# Autodesk Inventor assembly: ModuloCocina
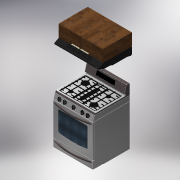
[picture p0: Inventor's stored thumbnail of the model, 180x180]
Saved by Autodesk Inventor 2016 (Build 200138000, 138)
## iProperties
Created: 2015-11-24
Part Number: ModuloCocina
Material: Genérico
Document SubType Name: Assembly
Designer: eolun
Author: eolun
## Documents named in this file (3)
- D:\Documents\Carrera\11.Semeste_II_2015\Computacion_grafica\Proyecto\COCINA_FINAL\Cocina\ModuloCocina.iam
- D:\Documents\Carrera\11.Semeste_II_2015\Computacion_grafica\Proyecto\COCINA_FINAL\Cocina\estufa.ipt
- D:\Documents\Carrera\11.Semeste_II_2015\Computacion_grafica\Proyecto\COCINA_FINAL\Cocina\ModuloExtractor.iam
## Components (2 placed, 2 different names)
1. estufa:1 — Nivelación:1, Nivelación:2, Coincidencia:1
2. ModuloExtractor:1 [sub-assembly] — Nivelación:1, Nivelación:2, Coincidencia:1
## Relationships (3: Flush 2, Mate 1)
- Nivelación:1 [Flush] (-44 mm): estufa:1 ↔ ModuloExtractor:1
- Nivelación:2 [Flush]: estufa:1 ↔ ModuloExtractor:1
- Coincidencia:1 [Mate] (-1600 mm): estufa:1 ↔ ModuloExtractor:1
